# Autodesk Inventor assembly: Assembly_Eyepiece_Folded_mirror_withfocus
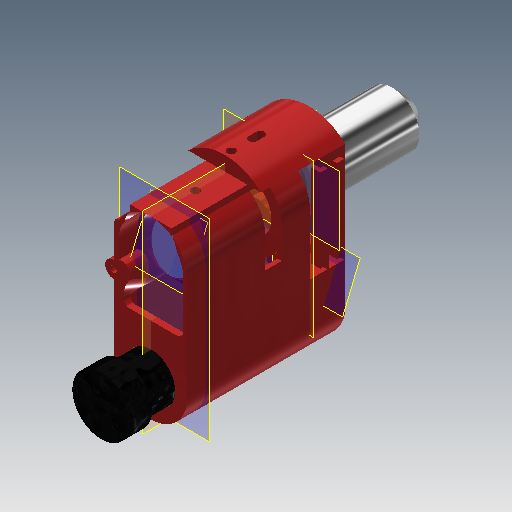
[picture p0: Inventor's stored thumbnail of the model, 512x512]
Saved by Autodesk Inventor 2019 (Build 230136000, 136)
## iProperties
Created: 2019-11-14
Part Number: Assembly_Eyepiece_Folded_mirror_withfocus
Document SubType Name: Assembly
Designer: diederichbenedict
Author: diederichbenedict
## Documents named in this file (6)
- C:\Users\diederichbenedict\Dropbox\Dokumente\Promotion\PROJECTS\STORMoChip\GITHUB\CAD\Nanoscopy-on-the-cheap\Workspace\Assembly_Eyepiece_Folded_mirror_withfocus.iam
- C:\Users\diederichbenedict\Dropbox\Dokumente\Promotion\PROJECTS\STORMoChip\GITHUB\CAD\Nanoscopy-on-the-cheap\Workspace\00_Eyepiece_20x_WF.ipt
- C:\Users\diederichbenedict\Dropbox\Dokumente\Promotion\PROJECTS\STORMoChip\GITHUB\CAD\Nanoscopy-on-the-cheap\Workspace\00_Microscope_Objective.ipt
- C:\Users\diederichbenedict\Dropbox\Dokumente\Promotion\PROJECTS\STORMoChip\GITHUB\CAD\Nanoscopy-on-the-cheap\Workspace\PF10-03-P01-Step.ipt
- C:\Users\diederichbenedict\Dropbox\Dokumente\Promotion\PROJECTS\STORMoChip\GITHUB\CAD\Nanoscopy-on-the-cheap\Workspace\cellSTORM_objective_tube_folded_mirror_v2_longtube_R1.ipt
- C:\Users\diederichbenedict\Dropbox\Dokumente\Promotion\PROJECTS\STORMoChip\GITHUB\CAD\Nanoscopy-on-the-cheap\Workspace\cellSTORM_objective_thread.ipt
## Components (6 placed, 5 different names)
1. cellSTORM_objective_tube_folded_mirror_v2_longtube_R1:1 — Mate:2, Angle:4, Insert:8, Insert:9, Insert:10
2. cellSTORM_objective_thread:1 — Mate:2, Angle:4, Insert:7
3. 00_Microscope_Objective:2 — Insert:7
4. 00_Eyepiece_20x_WF:2 — Insert:8
5. PF10-03-P01-Step:4 — Insert:10
6. PF10-03-P01-Step:5 — Insert:9
## Relationships (6: Insert 4, Mate 1, Angle 1)
- Mate:2: cellSTORM_objective_tube_folded_mirror_v2_longtube_R1:1 ↔ cellSTORM_objective_thread:1
- Angle:4 (0 deg): cellSTORM_objective_tube_folded_mirror_v2_longtube_R1:1 ↔ cellSTORM_objective_thread:1
- Insert:7: cellSTORM_objective_thread:1 ↔ 00_Microscope_Objective:2
- Insert:8: cellSTORM_objective_tube_folded_mirror_v2_longtube_R1:1 ↔ 00_Eyepiece_20x_WF:2
- Insert:9: cellSTORM_objective_tube_folded_mirror_v2_longtube_R1:1 ↔ PF10-03-P01-Step:5
- Insert:10: cellSTORM_objective_tube_folded_mirror_v2_longtube_R1:1 ↔ PF10-03-P01-Step:4
